# Autodesk Inventor assembly: Raspberry_Pi_Assemby
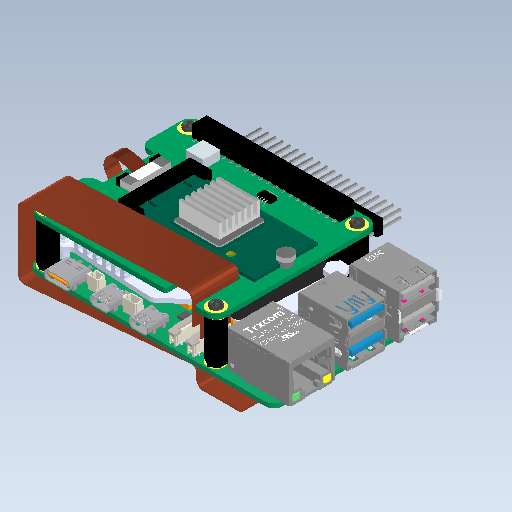
[picture p0: Inventor's stored thumbnail of the model, 512x512]
Saved by Autodesk Inventor 2021 (Build 250183000, 183)
## iProperties
Created: 2025-03-01
Part Number: Raspberry_Pi_Assemby
Document SubType Name: Assembly
Designer: 22liatho
Author: 22liatho
## Documents named in this file (7)
- C:\Users\22liatho\OneDrive - ABB Gymnasiet\Årskurs 3\Profil\Gymnasiearbete\GyArb Hållare CAD\CAD-filer\Raspberry_Pi_Assemby.iam
- C:\Users\22liatho\OneDrive - ABB Gymnasiet\Årskurs 3\Profil\Gymnasiearbete\GyArb Hållare CAD\raspberry-pi-5-2.snapshot.8\NEW STEP\Raspberry_Pi_5_Base.ipt
- C:\Users\22liatho\OneDrive - ABB Gymnasiet\Årskurs 3\Profil\Gymnasiearbete\GyArb Hållare CAD\CAD-filer\Raspberry_Pi_M.2_Hat+.ipt
- C:\Users\22liatho\OneDrive - ABB Gymnasiet\Årskurs 3\Profil\Gymnasiearbete\GyArb Hållare CAD\CAD-filer\Threaded_Pins.ipt
- C:\Users\22liatho\OneDrive - ABB Gymnasiet\Årskurs 3\Profil\Gymnasiearbete\GyArb Hållare CAD\CAD-filer\IO_Pin_Extension.ipt
- C:\Users\22liatho\OneDrive - ABB Gymnasiet\Årskurs 3\Profil\Gymnasiearbete\GyArb Hållare CAD\CAD-filer\Raspberry_Pi_Heatsink+fan.iam
- C:\Users\22liatho\Documents\Inventor\Content Center Files\R2021\en-US\ISO 7045(1)\DIN EN ISO 7045 - M2 x 3 - 4.8 - H.ipt
## Components (16 placed, 6 different names)
1. Raspberry_Pi_5_Base:1 — Mate:1, Mate:2, Mate:5, Flush:1, Flush:2, Mate:6, Mate:7, Mate:8, Mate:9, Mate:10, Mate:11, Mate:12, Mate:13, Mate:22, Mate:23, Mate:24, Mate:25, Mate:26, Mate:27, Mate:28, Mate:29
2. Raspberry_Pi_M.2_Hat+:1 — Mate:3, Mate:4, Mate:14, Mate:15, Mate:16, Mate:17, Mate:18, Mate:19, Mate:20, Mate:21, Mate:30
3. Threaded_Pins:1 — Mate:1, Mate:2, Mate:3, Mate:4
4. IO_Pin_Extension:1 — Mate:5, Flush:1, Flush:2
5. Threaded_Pins:2 — Mate:6, Mate:7, Mate:30
6. Threaded_Pins:3 — Mate:8, Mate:9
7. Threaded_Pins:4 — Mate:10, Mate:11
8. Raspberry_Pi_Heatsink+fan:1 [sub-assembly] — Mate:12, Mate:13
9. DIN EN ISO 7045 H M2 x 3 - 4.8 - H:1 — Mate:14, Mate:15
10. DIN EN ISO 7045 H M2 x 3 - 4.8 - H:2 — Mate:16, Mate:17
11. DIN EN ISO 7045 H M2 x 3 - 4.8 - H:3 — Mate:18, Mate:19
12. DIN EN ISO 7045 H M2 x 3 - 4.8 - H:4 — Mate:20, Mate:21
13. DIN EN ISO 7045 H M2 x 3 - 4.8 - H:5 — Mate:22, Mate:23
14. DIN EN ISO 7045 H M2 x 3 - 4.8 - H:6 — Mate:24, Mate:25
15. DIN EN ISO 7045 H M2 x 3 - 4.8 - H:7 — Mate:26, Mate:27
16. DIN EN ISO 7045 H M2 x 3 - 4.8 - H:8 — Mate:28, Mate:29
## Relationships (32: Mate 30, Flush 2)
- Mate:1: Raspberry_Pi_5_Base:1 ↔ Threaded_Pins:1
- Mate:2: Raspberry_Pi_5_Base:1 ↔ Threaded_Pins:1
- Mate:3: Raspberry_Pi_M.2_Hat+:1 ↔ Threaded_Pins:1
- Mate:4: Raspberry_Pi_M.2_Hat+:1 ↔ Threaded_Pins:1
- Mate:5: Raspberry_Pi_5_Base:1 ↔ IO_Pin_Extension:1
- Flush:1: Raspberry_Pi_5_Base:1 ↔ IO_Pin_Extension:1
- Flush:2: Raspberry_Pi_5_Base:1 ↔ IO_Pin_Extension:1
- Mate:6: Raspberry_Pi_5_Base:1 ↔ Threaded_Pins:2
- Mate:7: Raspberry_Pi_5_Base:1 ↔ Threaded_Pins:2
- Mate:8: Raspberry_Pi_5_Base:1 ↔ Threaded_Pins:3
- Mate:9: Raspberry_Pi_5_Base:1 ↔ Threaded_Pins:3
- Mate:10: Raspberry_Pi_5_Base:1 ↔ Threaded_Pins:4
- Mate:11: Raspberry_Pi_5_Base:1 ↔ Threaded_Pins:4
- Mate:12: Raspberry_Pi_5_Base:1 ↔ Raspberry_Pi_Heatsink+fan:1
- Mate:13: Raspberry_Pi_5_Base:1 ↔ Raspberry_Pi_Heatsink+fan:1
- Mate:14: Raspberry_Pi_M.2_Hat+:1 ↔ DIN EN ISO 7045 H M2 x 3 - 4.8 - H:1
- Mate:15: Raspberry_Pi_M.2_Hat+:1 ↔ DIN EN ISO 7045 H M2 x 3 - 4.8 - H:1
- Mate:16: Raspberry_Pi_M.2_Hat+:1 ↔ DIN EN ISO 7045 H M2 x 3 - 4.8 - H:2
- Mate:17: Raspberry_Pi_M.2_Hat+:1 ↔ DIN EN ISO 7045 H M2 x 3 - 4.8 - H:2
- Mate:18: Raspberry_Pi_M.2_Hat+:1 ↔ DIN EN ISO 7045 H M2 x 3 - 4.8 - H:3
- Mate:19: Raspberry_Pi_M.2_Hat+:1 ↔ DIN EN ISO 7045 H M2 x 3 - 4.8 - H:3
- Mate:20: Raspberry_Pi_M.2_Hat+:1 ↔ DIN EN ISO 7045 H M2 x 3 - 4.8 - H:4
- Mate:21: Raspberry_Pi_M.2_Hat+:1 ↔ DIN EN ISO 7045 H M2 x 3 - 4.8 - H:4
- Mate:22: Raspberry_Pi_5_Base:1 ↔ DIN EN ISO 7045 H M2 x 3 - 4.8 - H:5
- Mate:23: Raspberry_Pi_5_Base:1 ↔ DIN EN ISO 7045 H M2 x 3 - 4.8 - H:5
- Mate:24: Raspberry_Pi_5_Base:1 ↔ DIN EN ISO 7045 H M2 x 3 - 4.8 - H:6
- Mate:25: Raspberry_Pi_5_Base:1 ↔ DIN EN ISO 7045 H M2 x 3 - 4.8 - H:6
- Mate:26: Raspberry_Pi_5_Base:1 ↔ DIN EN ISO 7045 H M2 x 3 - 4.8 - H:7
- Mate:27: Raspberry_Pi_5_Base:1 ↔ DIN EN ISO 7045 H M2 x 3 - 4.8 - H:7
- Mate:28: Raspberry_Pi_5_Base:1 ↔ DIN EN ISO 7045 H M2 x 3 - 4.8 - H:8
- Mate:29: Raspberry_Pi_5_Base:1 ↔ DIN EN ISO 7045 H M2 x 3 - 4.8 - H:8
- Mate:30: Raspberry_Pi_M.2_Hat+:1 ↔ Threaded_Pins:2
